# Autodesk Inventor assembly: Hinge_Assy_54A08_15in
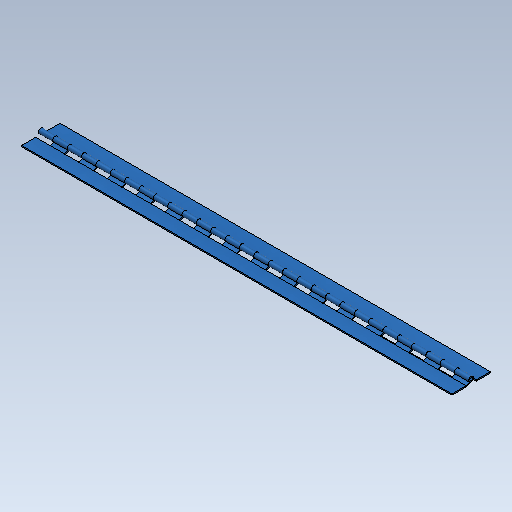
[picture p0: Inventor's stored thumbnail of the model, 512x512]
Saved by Autodesk Inventor 2020.1 (Build 241239000, 239)
## iProperties
Created: 2009-10-15
Part Number: Hinge_Assy_54A08_15in
Document SubType Name: Assembly
Designer: Thom Tremblay
Author: Thom Tremblay
## Documents named in this file (2)
- C:\Users\thom_tremblay\Desktop\Inventor ACP prep data\Week 1\Electrical Enclosure\Hinge.iam
- C:\Users\thom_tremblay\Desktop\Inventor ACP prep data\Week 1\Electrical Enclosure\hinge_barrel_54A08_15in.ipt
## Components (2 placed, 1 different names)
1. hinge_barrel_54A08_15in:1 — Insert:1
2. hinge_barrel_54A08_15in:2 — Insert:1
## Relationships (1: Insert 1)
- Insert:1: hinge_barrel_54A08_15in:1 ↔ hinge_barrel_54A08_15in:2
